# Autodesk Inventor assembly: y_axis
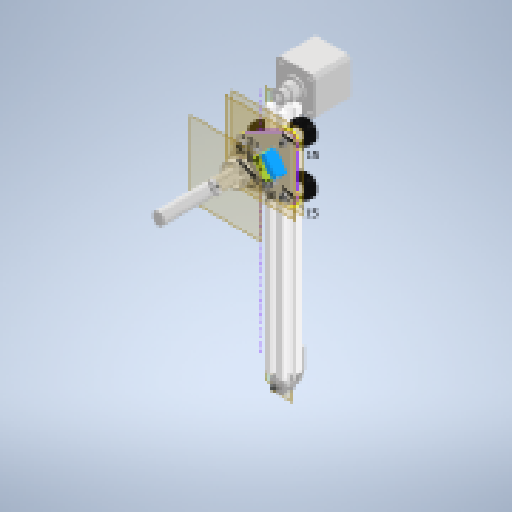
[picture p0: Inventor's stored thumbnail of the model, 512x512]
Saved by Autodesk Inventor 2024 (Build 280153000, 153)
## iProperties
Created: 2026-02-05
Part Number: y_axis
Document SubType Name: Assembly
Designer: SEMEN
Author: SEMEN
## Documents named in this file (25)
- C:\Users\SEMEN\Documents\ETZ2.0\y_axis.iam
- C:\Users\SEMEN\Documents\ETZ2.0\Alumunium T Profile 20x20, 100cm v3.ipt
- C:\Users\SEMEN\Documents\ETZ2.0\motor_x.ipt
- C:\Users\SEMEN\Documents\ETZ2.0\belt_gear_1.ipt
- C:\Users\SEMEN\Documents\ETZ2.0\belt_gear_2.ipt
- C:\Users\SEMEN\Documents\ETZ2.0\belt_tentioner_plane.ipt
- C:\Users\SEMEN\Documents\ETZ2.0\belt_tentioner_washer.ipt
- C:\Users\SEMEN\Documents\Inventor\Content Center Files\R2024\en-US\ISO 7046-1 H(1)\ISO 7046-1 - M5 x 25_ - 4.8 - H - ISO.ipt
- C:\Users\SEMEN\Documents\Inventor\Content Center Files\R2024\en-US\ISO 4032(2)\ISO 4032 - M5 - ISO.ipt
- C:\Users\SEMEN\Documents\Inventor\Content Center Files\R2024\en-US\ISO 7046-1 H(1)\ISO 7046-1 - M4 x 8_ - 4.8 - H - ISO.ipt
- C:\Users\SEMEN\Documents\ETZ2.0\profile_bearing.ipt
- C:\Users\SEMEN\Documents\ETZ2.0\plate_3.ipt
- C:\Users\SEMEN\Documents\Inventor\Content Center Files\R2024\en-US\ISO 7045  H\ISO 7045 - M4 x 30_ - 4.8 - H - ISO.ipt
- C:\Users\SEMEN\Documents\Inventor\Content Center Files\R2024\en-US\ISO 4032(2)\ISO 4032 - M4 - ISO.ipt
- C:\Users\SEMEN\Documents\ETZ2.0\plate_3_washers.ipt
- C:\Users\SEMEN\Documents\ETZ2.0\rail_holder.ipt
- C:\Users\SEMEN\Documents\ETZ2.0\rod.ipt
- C:\Users\SEMEN\Documents\Inventor\Content Center Files\R2024\en-US\ISO 7045  H\ISO 7045 - M2 x 8_ - 4.8 - H - ISO.ipt
- C:\Users\SEMEN\Documents\Inventor\Content Center Files\R2024\en-US\ISO 4032(2)\ISO 4032 - M2 - ISO.ipt
- C:\Users\SEMEN\Documents\ETZ2.0\spring.ipt
- C:\Users\SEMEN\Documents\ETZ2.0\marker_cerret.ipt
- C:\Users\SEMEN\Documents\Inventor\Content Center Files\R2024\en-US\ISO 7045  H\ISO 7045 - M4 x 16_ - 4.8 - H - ISO.ipt
- C:\Users\SEMEN\Documents\ETZ2.0\marker.ipt
- C:\Users\SEMEN\Documents\ETZ2.0\SG90_Servo_Motor.ipt
- C:\Users\SEMEN\Documents\ETZ2.0\servo_holder.ipt
## Components (41 placed, 24 different names)
1. motor_y:1 — Mate:1, Mate:2, Angle:1
2. Alumunium T Profile 20x20, 100cm v3:1 — Tangent:1, Flush:1, Mate:2, Angle:1, Tangent:2, Flush:2, Tangent:3, Tangent:4, Flush:3, Flush:4, Tangent:5, Mate:8, Mate:9, Tangent:6, Tangent:7, Mate:10, Mate:14
3. belt_gear_1:1 — Mate:1, Tangent:1, Flush:1, Tangent:2
4. belt_gear_2:1 — Flush:2, Tangent:3, Tangent:4, Mate:5
5. belt_tentioner_plane:1 — Flush:3, Flush:4, Flush:5, Mate:3, Mate:4, Mate:6, Mate:7
6. belt_tentioner_washer:1 — Flush:5
7. profile_bearing:1 — Tangent:5, Mate:8, Mate:11, Mate:12, Mate:29, Mate:35, Mate:36
8. profile_bearing:2 — Mate:9, Tangent:6, Mate:12, Mate:13, Mate:31, Mate:39, Mate:40
9. profile_bearing:3 — Tangent:7, Mate:10, Mate:11, Mate:13, Mate:37, Mate:38
10. plate_3:1 — Mate:14, Mate:33, Mate:42, Mate:44, Mate:46, Mate:47, Mate:51, Flush:6, Mate:53, Mate:54, Mate:55, Mate:56, Mate:57, Mate:67, Mate:77, Mate:79
11. plate_3_washers:1 — Mate:29, Mate:52
12. plate_3_washers:3 — Mate:33, Mate:50
13. plate_3_washers:2 — Mate:31, Mate:48
14. ISO 7046-1 H M5 x 25 - 4.8 - H:1 — Mate:3
15. ISO 4032 M5:1 — Mate:4, Mate:5
16. ISO 7046-1 H M4 x 8 - 4.8 - H:1 — Mate:6
17. ISO 7046-1 H M4 x 8 - 4.8 - H:2 — Mate:7
18. ISO 7045 H M4 x 30 - 4.8 - H:1 — Mate:35, Mate:36, Mate:43, Mate:52
19. ISO 7045 H M4 x 30 - 4.8 - H:2 — Mate:37, Mate:38, Mate:45, Mate:47, Mate:50
20. ISO 7045 H M4 x 30 - 4.8 - H:3 — Mate:39, Mate:40, Mate:41, Mate:48, Mate:51
21. ISO 4032 M4:1 — Mate:41, Mate:42
22. ISO 4032 M4:2 — Mate:43, Mate:44
23. ISO 4032 M4:3 — Mate:45, Mate:46
24. rail_holder:1 — Flush:6, Mate:58, Mate:59, Mate:60, Mate:61, Mate:67, Tangent:10
25. rail_holder:2 — Mate:53, Mate:54, Mate:55, Flush:7, Flush:8, Mate:62, Mate:63, Mate:64, Mate:65
26. rod:1 — Mate:56, Flush:7, Mate:69, Mate:71
27. rod:2 — Mate:57, Flush:8, Mate:66, Mate:70, Flush:9
28. ISO 7045 H M2 x 8 - 4.8 - H:1 — Mate:58, Mate:59
29. ISO 4032 M2:1 — Mate:60, Mate:61
30. ISO 7045 H M2 x 8 - 4.8 - H:2 — Mate:62, Mate:63
31. ISO 4032 M2:2 — Mate:64, Mate:65
32. spring:1 — Mate:66
33. spring:2 — Mate:69
34. marker_cerret:1 — Mate:76, Tangent:8, Tangent:9, Mate:78, Flush:10
35. rail_holder:3 — Mate:70, Mate:71, Flush:9, Mate:72, Mate:73, Mate:74, Mate:75
36. ISO 7045 H M2 x 8 - 4.8 - H:3 — Mate:72, Mate:73
37. ISO 4032 M2:3 — Mate:74, Mate:75
38. ISO 7045 H M4 x 16 - 4.8 - H:1 — Mate:76
39. marker:1 — Tangent:8, Tangent:9
40. SG90_Servo_Motor:1 — Mate:77, Mate:78, Tangent:10, Flush:10
41. servo_holder:1 — Mate:79
## Relationships (81: Mate 60, Tangent 10, Flush 10, Angle 1)
- Mate:1: motor_y:1 ↔ belt_gear_1:1
- Tangent:1 (1 mm): Alumunium T Profile 20x20, 100cm v3:1 ↔ belt_gear_1:1
- Flush:1 (0.5 mm): Alumunium T Profile 20x20, 100cm v3:1 ↔ belt_gear_1:1
- Mate:2 (4 mm): motor_y:1 ↔ Alumunium T Profile 20x20, 100cm v3:1
- Angle:1 (0 deg): motor_y:1 ↔ Alumunium T Profile 20x20, 100cm v3:1
- Tangent:2 (2 mm): Alumunium T Profile 20x20, 100cm v3:1 ↔ belt_gear_1:1
- Flush:2 (0.7 mm): Alumunium T Profile 20x20, 100cm v3:1 ↔ belt_gear_2:1
- Tangent:3 (1 mm): Alumunium T Profile 20x20, 100cm v3:1 ↔ belt_gear_2:1
- Tangent:4 (1 mm): Alumunium T Profile 20x20, 100cm v3:1 ↔ belt_gear_2:1
- Flush:3: Alumunium T Profile 20x20, 100cm v3:1 ↔ belt_tentioner_plane:1
- Flush:4: Alumunium T Profile 20x20, 100cm v3:1 ↔ belt_tentioner_plane:1
- Flush:5: belt_tentioner_plane:1 ↔ belt_tentioner_washer:1
- Mate:3: belt_tentioner_plane:1 ↔ ISO 7046-1 H M5 x 25 - 4.8 - H:1
- Mate:4: belt_tentioner_plane:1 ↔ ISO 4032 M5:1
- Mate:5: belt_gear_2:1 ↔ ISO 4032 M5:1
- Mate:6: belt_tentioner_plane:1 ↔ ISO 7046-1 H M4 x 8 - 4.8 - H:1
- Mate:7: belt_tentioner_plane:1 ↔ ISO 7046-1 H M4 x 8 - 4.8 - H:2
- Tangent:5: Alumunium T Profile 20x20, 100cm v3:1 ↔ profile_bearing:1
- Mate:8 (-2 mm): Alumunium T Profile 20x20, 100cm v3:1 ↔ profile_bearing:1
- Mate:9 (-2 mm): Alumunium T Profile 20x20, 100cm v3:1 ↔ profile_bearing:2
- Tangent:6: Alumunium T Profile 20x20, 100cm v3:1 ↔ profile_bearing:2
- Tangent:7: Alumunium T Profile 20x20, 100cm v3:1 ↔ profile_bearing:3
- Mate:10 (-2 mm): Alumunium T Profile 20x20, 100cm v3:1 ↔ profile_bearing:3
- Mate:11 (50.8068 mm): profile_bearing:1 ↔ profile_bearing:3
- Mate:12 (50.8068 mm): profile_bearing:1 ↔ profile_bearing:2
- Mate:13 (50.8068 mm): profile_bearing:2 ↔ profile_bearing:3
- Mate:14 (5 mm): Alumunium T Profile 20x20, 100cm v3:1 ↔ plate_3:1
- Mate:29: profile_bearing:1 ↔ plate_3_washers:1
- Mate:31: profile_bearing:2 ↔ plate_3_washers:2
- Mate:33: plate_3:1 ↔ plate_3_washers:3
- Mate:35: profile_bearing:1 ↔ ISO 7045 H M4 x 30 - 4.8 - H:1
- Mate:36: profile_bearing:1 ↔ ISO 7045 H M4 x 30 - 4.8 - H:1
- Mate:37: profile_bearing:3 ↔ ISO 7045 H M4 x 30 - 4.8 - H:2
- Mate:38: profile_bearing:3 ↔ ISO 7045 H M4 x 30 - 4.8 - H:2
- Mate:39: profile_bearing:2 ↔ ISO 7045 H M4 x 30 - 4.8 - H:3
- Mate:40: profile_bearing:2 ↔ ISO 7045 H M4 x 30 - 4.8 - H:3
- Mate:41: ISO 7045 H M4 x 30 - 4.8 - H:3 ↔ ISO 4032 M4:1
- Mate:42: plate_3:1 ↔ ISO 4032 M4:1
- Mate:43: ISO 7045 H M4 x 30 - 4.8 - H:1 ↔ ISO 4032 M4:2
- Mate:44: plate_3:1 ↔ ISO 4032 M4:2
- Mate:45: ISO 7045 H M4 x 30 - 4.8 - H:2 ↔ ISO 4032 M4:3
- Mate:46: plate_3:1 ↔ ISO 4032 M4:3
- Mate:47: plate_3:1 ↔ ISO 7045 H M4 x 30 - 4.8 - H:2
- Mate:48: plate_3_washers:2 ↔ ISO 7045 H M4 x 30 - 4.8 - H:3
- Mate:50: plate_3_washers:3 ↔ ISO 7045 H M4 x 30 - 4.8 - H:2
- Mate:51: plate_3:1 ↔ ISO 7045 H M4 x 30 - 4.8 - H:3
- Mate:52: plate_3_washers:1 ↔ ISO 7045 H M4 x 30 - 4.8 - H:1
- Flush:6: plate_3:1 ↔ rail_holder:1
- Mate:53: plate_3:1 ↔ rail_holder:2
- Mate:54: plate_3:1 ↔ rail_holder:2
- Mate:55: plate_3:1 ↔ rail_holder:2
- Mate:56: plate_3:1 ↔ rod:1
- Flush:7: rail_holder:2 ↔ rod:1
- Mate:57: plate_3:1 ↔ rod:2
- Flush:8: rail_holder:2 ↔ rod:2
- Mate:58: rail_holder:1 ↔ ISO 7045 H M2 x 8 - 4.8 - H:1
- Mate:59: rail_holder:1 ↔ ISO 7045 H M2 x 8 - 4.8 - H:1
- Mate:60: rail_holder:1 ↔ ISO 4032 M2:1
- Mate:61: rail_holder:1 ↔ ISO 4032 M2:1
- Mate:62: rail_holder:2 ↔ ISO 7045 H M2 x 8 - 4.8 - H:2
- Mate:63: rail_holder:2 ↔ ISO 7045 H M2 x 8 - 4.8 - H:2
- Mate:64: rail_holder:2 ↔ ISO 4032 M2:2
- Mate:65: rail_holder:2 ↔ ISO 4032 M2:2
- Mate:66: rod:2 ↔ spring:1
- Mate:67: plate_3:1 ↔ rail_holder:1
- Mate:69: rod:1 ↔ spring:2
- Mate:70: rod:2 ↔ rail_holder:3
- Mate:71: rod:1 ↔ rail_holder:3
- Flush:9: rod:2 ↔ rail_holder:3
- Mate:72: rail_holder:3 ↔ ISO 7045 H M2 x 8 - 4.8 - H:3
- Mate:73: rail_holder:3 ↔ ISO 7045 H M2 x 8 - 4.8 - H:3
- Mate:74: rail_holder:3 ↔ ISO 4032 M2:3
- Mate:75: rail_holder:3 ↔ ISO 4032 M2:3
- Mate:76: marker_cerret:1 ↔ ISO 7045 H M4 x 16 - 4.8 - H:1
- Tangent:8: marker_cerret:1 ↔ marker:1
- Tangent:9: marker_cerret:1 ↔ marker:1
- Mate:77: plate_3:1 ↔ SG90_Servo_Motor:1
- Mate:78 (2 mm): marker_cerret:1 ↔ SG90_Servo_Motor:1
- Mate:79: plate_3:1 ↔ servo_holder:1
- Tangent:10 (-10 mm): rail_holder:1 ↔ SG90_Servo_Motor:1
- Flush:10: marker_cerret:1 ↔ SG90_Servo_Motor:1
